# Autodesk Inventor assembly: main
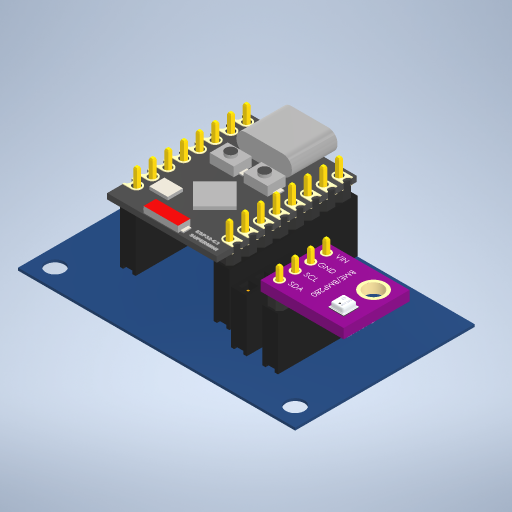
[picture p0: Inventor's stored thumbnail of the model, 512x512]
Saved by Autodesk Inventor 2024 (Build 280153000, 153)
## iProperties
Created: 2025-04-09
Part Number: main
Document SubType Name: Assembly
Designer: erikt
Author: erikt
## Documents named in this file (8)
- C:\HTL\4AHEL\PBE\PBE_KuenC\Umgebungssensor\Gehaeuse_Umgebungssensor\main.iam
- C:\HTL\4AHEL\PBE\PBE_KuenC\Umgebungssensor\Gehaeuse_Umgebungssensor\Umgebungssensor_PCB\Umgebungssensor_PCB.ipt
- C:\HTL\4AHEL\PBE\PBE_KuenC\Umgebungssensor\Gehaeuse_Umgebungssensor\zl262-4s_p2-54_l10-6_w2-54_h8-5\zl262-4s_p2-54_l10-6_w2-54_h8-5.ipt
- C:\HTL\4AHEL\PBE\PBE_KuenC\Umgebungssensor\Gehaeuse_Umgebungssensor\zl262-8s_p2-54_l20-8_w2-54_h8-5\zl262-8s_p2-54_l20-8_w2-54_h8-5.ipt
- C:\HTL\4AHEL\PBE\PBE_KuenC\Umgebungssensor\Gehaeuse_Umgebungssensor\ESP32-C3 supermini v5\ESP32-C3 supermini v5.ipt
- C:\HTL\4AHEL\PBE\PBE_KuenC\Umgebungssensor\Gehaeuse_Umgebungssensor\PLS-8\PLS-8.ipt
- C:\HTL\4AHEL\PBE\PBE_KuenC\Umgebungssensor\Gehaeuse_Umgebungssensor\GY-BME280\GY-BME280.ipt
- C:\HTL\4AHEL\PBE\PBE_KuenC\Umgebungssensor\Gehaeuse_Umgebungssensor\PLS-4\PLS-4.ipt
## Components (10 placed, 7 different names)
1. Umgebungssensor_PCB:1 — Starr:1, Starr:2, Starr:3, Starr:4
2. zl262-4s_p2-54_l10-6_w2-54_h8-5:1 — Starr:1
3. zl262-4s_p2-54_l10-6_w2-54_h8-5:2 — Starr:2, Starr:9
4. zl262-8s_p2-54_l20-8_w2-54_h8-5:1 — Starr:4
5. zl262-8s_p2-54_l20-8_w2-54_h8-5:2 — Starr:3, Starr:7
6. GY-BME280:1 — Starr:8
7. PLS-4:1 — Starr:8, Starr:9
8. ESP32-C3 supermini v5:2 — Starr:5, Starr:6
9. PLS-8:1 — Starr:5, Starr:7
10. PLS-8:2 — Starr:6
## Relationships (9: WeldJoint 9)
- Starr:1 [WeldJoint] (-3 mm): Umgebungssensor_PCB:1 ↔ zl262-4s_p2-54_l10-6_w2-54_h8-5:1
- Starr:2 [WeldJoint] (2.589 mm): Umgebungssensor_PCB:1 ↔ zl262-4s_p2-54_l10-6_w2-54_h8-5:2
- Starr:3 [WeldJoint] (-3 mm): Umgebungssensor_PCB:1 ↔ zl262-8s_p2-54_l20-8_w2-54_h8-5:2
- Starr:4 [WeldJoint] (-3 mm): Umgebungssensor_PCB:1 ↔ zl262-8s_p2-54_l20-8_w2-54_h8-5:1
- Starr:5 [WeldJoint] (-2.7 mm): ESP32-C3 supermini v5:2 ↔ PLS-8:1
- Starr:6 [WeldJoint] (2.7 mm): ESP32-C3 supermini v5:2 ↔ PLS-8:2
- Starr:7 [WeldJoint] (1.5 mm): zl262-8s_p2-54_l20-8_w2-54_h8-5:2 ↔ PLS-8:1
- Starr:8 [WeldJoint] (2.09 mm): GY-BME280:1 ↔ PLS-4:1
- Starr:9 [WeldJoint] (1.5 mm): zl262-4s_p2-54_l10-6_w2-54_h8-5:2 ↔ PLS-4:1
